# Autodesk Inventor assembly: 547859 SMT-8G-PS-24V-E-2,5Q-OE
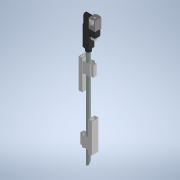
[picture p0: Inventor's stored thumbnail of the model, 180x180]
Saved by Autodesk Inventor 2021 (Build 250183000, 183)
## iProperties
Category: PARTsolutions
Company: FESTO
Created: 2025-06-24
Part Number: 547859 SMT-8G-PS-24V-E-2,5Q-OE
Catalog Web Link: www.cadenas.de
Description: SMT-proximity sensor
Vendor: FESTO
Document SubType Name: Assembly
Designer: psAdmin
Manufacturer: FESTO
Mass: 30 g
Surface Area: 37.3203 cm^2
Volume: 1.93696 cm^3
Density: 15.4882 g/cm^3
Title: 547859 SMT-8G-PS-24V-E-2,5Q-OE
Author: Cadenas PARTsolutions
Comments: proximity sensor
PSOL_IDENT_0: {ATYP=ASSISTANT},{DATA=script=$CADENAS_DATA/23d-libs/festo/webfesto.vbb&M_FAMILY=SMT&M_GROUP=01&M_PA
PSOL_IDENT_1: RTNO=547859&IDCODE1=SMT-8G-PS-24V-E-25Q-OE&IDCODE2=&customer_number_cns=&MATES=1&LOD=HI&LOCKERP=0&SI
PSOL_IDENT_2: NGLEPART=1}
NB: 547859 SMT-8G-PS-24V-E-2,5Q-OE
NN: SMT
NT: proximity sensor
NBSYN: $TNR. $TYP.
LINA: 547859 SMT-8G-PS-24V-E-2,5Q-OE
CATALOG: Festo
TNR: 547859
TYP: SMT-8G-PS-24V-E-2,5Q-OE
CNSMASSEXACT: 0.03
GTIN: 4052568093013
SUPPLIER: FESTO
ARTICLENO: 547859 SMT-8G-PS-24V-E-2,5Q-OE
BOMINFO: 547859 SMT-8G-PS-24V-E-2,5Q-OE
CREATOR: CADENAS GmbH
## Documents named in this file (3)
- e:\temp\worker_COMMON_242\temp\tmp_8392_106_wy5ST\format_0\547859 SMT-8G-PS-24V-E-2,5Q-OE.iam
- e:\temp\worker_COMMON_242\temp\tmp_8392_106_wy5ST\format_0\547859 SMT-8G-PS-24V-E-2,5Q-OE_G.ipt
- e:\temp\worker_COMMON_242\temp\tmp_8392_106_wy5ST\format_0\1247168 ASCF-M-23-S DM 2_1-3_4.ipt
## Components (3 placed, 2 different names)
1. 547859 SMT-8G-PS-24V-E-2,5Q-OE_G:1 — KTN1_XY@1 <-> KTN_XY@2, KTN1_Z@1 <-> KTN_Z@2, KTN1_YZ@1 <-> KTN_YZ@2, KTN2_XY@1 <-> KTN_XY@3, KTN2_Z@1 <-> KTN_Z@3, KTN2_YZ@1 <-> KTN_YZ@3
2. 1247168 ASCF-M-23-S DM 2_1-3_4:1 — KTN1_XY@1 <-> KTN_XY@2, KTN1_Z@1 <-> KTN_Z@2, KTN1_YZ@1 <-> KTN_YZ@2
3. 1247168 ASCF-M-23-S DM 2_1-3_4:2 — KTN2_XY@1 <-> KTN_XY@3, KTN2_Z@1 <-> KTN_Z@3, KTN2_YZ@1 <-> KTN_YZ@3
## Relationships (6: Mate 4, Angle 2)
- KTN1_XY@1 <-> KTN_XY@2 [Mate]: 547859 SMT-8G-PS-24V-E-2,5Q-OE_G:1 ↔ 1247168 ASCF-M-23-S DM 2_1-3_4:1
- KTN1_Z@1 <-> KTN_Z@2 [Mate]: 547859 SMT-8G-PS-24V-E-2,5Q-OE_G:1 ↔ 1247168 ASCF-M-23-S DM 2_1-3_4:1
- KTN1_YZ@1 <-> KTN_YZ@2 [Angle] (0 deg): 547859 SMT-8G-PS-24V-E-2,5Q-OE_G:1 ↔ 1247168 ASCF-M-23-S DM 2_1-3_4:1
- KTN2_XY@1 <-> KTN_XY@3 [Mate]: 547859 SMT-8G-PS-24V-E-2,5Q-OE_G:1 ↔ 1247168 ASCF-M-23-S DM 2_1-3_4:2
- KTN2_Z@1 <-> KTN_Z@3 [Mate]: 547859 SMT-8G-PS-24V-E-2,5Q-OE_G:1 ↔ 1247168 ASCF-M-23-S DM 2_1-3_4:2
- KTN2_YZ@1 <-> KTN_YZ@3 [Angle] (0 deg): 547859 SMT-8G-PS-24V-E-2,5Q-OE_G:1 ↔ 1247168 ASCF-M-23-S DM 2_1-3_4:2
